# Autodesk Inventor assembly: Shifter v4
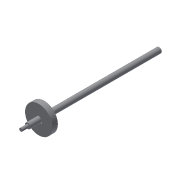
[picture p0: Inventor's stored thumbnail of the model, 180x180]
Saved by Autodesk Inventor 2014 (Build 180170000, 170)
## iProperties
Created: 2014-03-01
Part Number: Shifter v4
Document SubType Name: Assembly
Designer: Owner
Author: Owner
## Documents named in this file (5)
- C:\Users\Owner\Documents\Inventor\FRC 2014\Frc Chassis 2014\Shifter v4.iam
- C:\Users\Owner\Documents\Inventor\FRC 2014\Frc Chassis 2014\transmission tube v1.ipt
- C:\Users\Owner\Documents\Inventor\FRC 2014\Frc Chassis 2014\transmission plunger.ipt
- C:\Users\Owner\Documents\Inventor\FRC 2014\Frc Chassis 2014\Ball bearing - .1875.ipt
- C:\Users\Owner\Documents\Inventor\FRC 2014\Frc Chassis 2014\augmented gear v4.ipt
## Components (6 placed, 4 different names)
1. transmission tube v1:1 — Insert:1, Tangent:1, Tangent:2, Tangent:3, Tangent:9, Tangent:10
2. transmission plunger:1 — Insert:1, Tangent:6, Tangent:7, Tangent:8
3. Ball bearing - .1875:1 — Tangent:1, Tangent:7
4. Ball bearing - .1875:2 — Tangent:3, Tangent:8
5. Ball bearing - .1875:3 — Tangent:2, Tangent:6
6. augmented gear v4:1 — Tangent:9, Tangent:10
## Relationships (9: Tangent 8, Insert 1)
- Insert:1 (-12.7 mm): transmission tube v1:1 ↔ transmission plunger:1
- Tangent:1: transmission tube v1:1 ↔ Ball bearing - .1875:1
- Tangent:2: transmission tube v1:1 ↔ Ball bearing - .1875:3
- Tangent:3: transmission tube v1:1 ↔ Ball bearing - .1875:2
- Tangent:6: transmission plunger:1 ↔ Ball bearing - .1875:3
- Tangent:7: transmission plunger:1 ↔ Ball bearing - .1875:1
- Tangent:8: transmission plunger:1 ↔ Ball bearing - .1875:2
- Tangent:9: transmission tube v1:1 ↔ augmented gear v4:1
- Tangent:10: transmission tube v1:1 ↔ augmented gear v4:1
